# Autodesk Inventor assembly: 10 cell
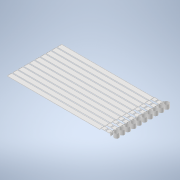
[picture p0: Inventor's stored thumbnail of the model, 180x180]
Saved by Autodesk Inventor 2020 (Build 240168000, 168)
## iProperties
Created: 2019-09-26
Part Number: 10 cell
Document SubType Name: Assembly
Designer: Abbas
Author: Abbas
## Documents named in this file (2)
- D:\Projects\aquaponic\Inventor\10 cell.iam
- D:\Projects\aquaponic\Inventor\1 cell.iam
## Components (10 placed, 1 different names)
1. 1 cell:1 [sub-assembly] — Mate:1
2. 1 cell:2 [sub-assembly]
3. 1 cell:3 [sub-assembly]
4. 1 cell:4 [sub-assembly]
5. 1 cell:5 [sub-assembly]
6. 1 cell:6 [sub-assembly]
7. 1 cell:7 [sub-assembly]
8. 1 cell:8 [sub-assembly]
9. 1 cell:9 [sub-assembly]
10. 1 cell:10 [sub-assembly]
## Component patterns: (10 elements, first: 1 cell:1)
## Relationships (1: Mate 1)
- Mate:1: 1 cell:1
